# Autodesk Inventor assembly: PC-Dummie
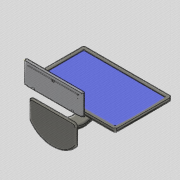
[picture p0: Inventor's stored thumbnail of the model, 180x180]
Saved by Autodesk Inventor 2018.2 (Build 222227000, 227)
## iProperties
Company: Fraunhofer ILT
Created: 2018-11-08
Part Number: PC-Dummie
Material: geeigneten Werkstoff auswählen !
Document SubType Name: Assembly
Designer: N.Grubert
Title: =Description
Author: N.Grubert
## Documents named in this file (3)
- V:\A340\2018\DOKUMENTATION\COSIMA\COSIMA-Laserstar\CAD\Computer-Dummie\PC-Dummie.iam
- V:\A340\2018\DOKUMENTATION\COSIMA\COSIMA-Laserstar\CAD\Computer-Dummie\Monitor.ipt
- V:\A340\2018\DOKUMENTATION\COSIMA\COSIMA-Laserstar\CAD\Computer-Dummie\Tastatur.ipt
## Components (2 placed, 2 different names)
1. Monitor:1 — Fluchtend:1
2. Tastatur:1 — Fluchtend:1
## Relationships (1: Flush 1)
- Fluchtend:1 [Flush]: Monitor:1 ↔ Tastatur:1
